# Autodesk Inventor assembly: ShooterAssemblyV05
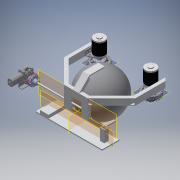
[picture p0: Inventor's stored thumbnail of the model, 180x180]
Saved by Autodesk Inventor 2016 SP1 (Build 200210100, 210)
## iProperties
Created: 2016-02-07
Part Number: ShooterAssemblyV05
Document SubType Name: Assembly
Designer: steele
Author: steele
## Documents named in this file (12)
- C:\snobotics\CAD-Development\robSteele\SnoBotics2016\2016-05-05-ShooterPrototype\ShooterAssemblyV05.iam
- C:\snobotics\CAD-Development\robSteele\SnoBotics2016\DraftOfBoulder.ipt
- C:\snobotics\CAD-Development\robSteele\SnoBotics2016\2016-05-05-ShooterPrototype\Mini_CIM_MotorHub_4_inch_wheel.iam
- C:\snobotics\CAD-Development\robSteele\SnoBotics2016\2016-05-05-ShooterPrototype\AluminumRodForShooter.ipt
- C:\snobotics\CAD-Development\robSteele\SnoBotics2016\AM Parts\SnowBlowerMotorAndHub.iam
- C:\snobotics\CAD-Development\robSteele\SnoBotics2016\AM Parts\rsSnowBlowerMount.ipt
- C:\snobotics\CAD-Development\robSteele\SnoBotics2016\2016-05-05-ShooterPrototype\SupportPlateToAttachToRobotBase.ipt
- C:\snobotics\CAD-Development\robSteele\SnoBotics2016\2016-05-05-ShooterPrototype\CIM_MotorHub_4_inch_wheel.iam
- C:\snobotics\CAD-Development\robSteele\SnoBotics2016\2016-05-05-ShooterPrototype\ShooterFrameAssembly05.iam
- C:\snobotics\CAD-Development\robSteele\SnoBotics2016\AM Parts\am-0134a+375+Key+Hub+r2.ipt
- C:\snobotics\CAD-Development\robSteele\SnoBotics2016\2016-05-05-ShooterPrototype\capForPost.ipt
- C:\snobotics\CAD-Development\robSteele\SnoBotics2016\2016-05-05-ShooterPrototype\ShooterAssemblyV05\Design Accelerator\Bolted Connection1.iam
## Components (11 placed, 11 different names)
1. ShooterFrameAssembly05:1 [sub-assembly] — Mate:1, Mate:16, Flush:6, Mate:17, Insert:4, Flush:9, Flush:10, Flush:11
2. Mini_CIM_MotorHub_4_inch_wheel:1 [sub-assembly] — Mate:1, Mate:3, Flush:5, Mate:16, Flush:6, Flush:7, Flush:8
3. DraftOfBoulder:1 — Mate:3, Flush:9
4. AluminumRodForShooter:1 — Insert:4, Insert:5
5. SnowBlowerMotorAndHub:1 [sub-assembly] — Mate:18, Insert:6, Mate:19
6. CIM_MotorHub_4_inch_wheel:1 [sub-assembly] — Flush:5, Mate:17, Flush:7, Flush:8
7. rsSnowBlowerMount:1 — Insert:6
8. SupportPlateToAttachToRobotBase:1 — Flush:10, Flush:11
9. am-0134a+375+Key+Hub+r2:1 — Insert:5, Mate:18, Mate:19
10. capForPost:1 — Mate:25, Mate:26
11. Bolted Connection:1 [sub-assembly] — Mate:25, Mate:26
## Relationships (18: Mate 8, Flush 7, Insert 3)
- Mate:1: ShooterFrameAssembly05:1 ↔ Mini_CIM_MotorHub_4_inch_wheel:1
- Mate:3: Mini_CIM_MotorHub_4_inch_wheel:1 ↔ DraftOfBoulder:1
- Flush:5: Mini_CIM_MotorHub_4_inch_wheel:1 ↔ CIM_MotorHub_4_inch_wheel:1
- Mate:16: ShooterFrameAssembly05:1 ↔ Mini_CIM_MotorHub_4_inch_wheel:1
- Flush:6 (-4.7625 mm): ShooterFrameAssembly05:1 ↔ Mini_CIM_MotorHub_4_inch_wheel:1
- Mate:17: ShooterFrameAssembly05:1 ↔ CIM_MotorHub_4_inch_wheel:1
- Flush:7: Mini_CIM_MotorHub_4_inch_wheel:1 ↔ CIM_MotorHub_4_inch_wheel:1
- Flush:8: Mini_CIM_MotorHub_4_inch_wheel:1 ↔ CIM_MotorHub_4_inch_wheel:1
- Insert:4: ShooterFrameAssembly05:1 ↔ AluminumRodForShooter:1
- Insert:5: AluminumRodForShooter:1 ↔ am-0134a+375+Key+Hub+r2:1
- Mate:18: SnowBlowerMotorAndHub:1 ↔ am-0134a+375+Key+Hub+r2:1
- Insert:6: SnowBlowerMotorAndHub:1 ↔ rsSnowBlowerMount:1
- Mate:19: SnowBlowerMotorAndHub:1 ↔ am-0134a+375+Key+Hub+r2:1
- Flush:9: ShooterFrameAssembly05:1 ↔ DraftOfBoulder:1
- Mate:25: capForPost:1 ↔ Bolted Connection:1
- Mate:26: capForPost:1 ↔ Bolted Connection:1
- Flush:10: ShooterFrameAssembly05:1 ↔ SupportPlateToAttachToRobotBase:1
- Flush:11: ShooterFrameAssembly05:1 ↔ SupportPlateToAttachToRobotBase:1
